# Autodesk Inventor assembly: Ensemble1
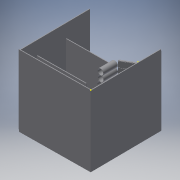
[picture p0: Inventor's stored thumbnail of the model, 180x180]
Saved by Autodesk Inventor 2019 (Build 230136000, 136)
## iProperties
Created: 2018-11-20
Part Number: Ensemble1
Material: Générique
Document SubType Name: Assembly
Designer: pouey
Author: pouey
## Documents named in this file (6)
- C:\Users\pouey\Desktop\PROJET ARDUINO\Ensemble1.iam
- C:\Users\pouey\Desktop\PROJET ARDUINO\boite.ipt
- C:\Users\pouey\Desktop\PROJET ARDUINO\V1.0_11-18.ipt
- C:\Users\pouey\Desktop\PROJET ARDUINO\planche.ipt
- C:\Users\pouey\Desktop\PROJET ARDUINO\toboggan.ipt
- C:\Users\pouey\Desktop\PROJET ARDUINO\tube.ipt
## Components (11 placed, 5 different names)
1. boite:1 — Placage:2, Placage:3, Placage:6, Placage:9, Placage:10, Placage:12, Placage:13, Placage:15, Placage:16, Placage:18, Angle:1
2. V1.0_11-18:1 — Placage:15, Placage:16
3. planche:1 — Placage:2, Placage:3, Placage:10, Placage:11
4. planche:2 — Placage:6, Placage:9, Placage:11, Placage:14
5. planche:3 — Placage:12, Placage:13, Placage:14
6. toboggan:1 — Placage:18, Angle:1, Placage:19, Placage:20, Placage:21, Placage:22, Placage:23
7. tube:1 — Placage:19
8. tube:2 — Placage:20
9. tube:3 — Placage:21
10. tube:4 — Placage:22
11. tube:5 — Placage:23
## Relationships (18: Mate 17, Angle 1)
- Placage:2 [Mate]: boite:1 ↔ planche:1
- Placage:3 [Mate] (120 mm): boite:1 ↔ planche:1
- Placage:6 [Mate]: boite:1 ↔ planche:2
- Placage:9 [Mate]: boite:1 ↔ planche:2
- Placage:10 [Mate]: boite:1 ↔ planche:1
- Placage:11 [Mate] (200 mm): planche:1 ↔ planche:2
- Placage:12 [Mate]: boite:1 ↔ planche:3
- Placage:13 [Mate]: boite:1 ↔ planche:3
- Placage:14 [Mate]: planche:2 ↔ planche:3
- Placage:15 [Mate]: boite:1 ↔ V1.0_11-18:1
- Placage:16 [Mate] (280 mm): boite:1 ↔ V1.0_11-18:1
- Placage:18 [Mate] (280 mm): boite:1 ↔ toboggan:1
- Angle:1 (120 deg): boite:1 ↔ toboggan:1
- Placage:19 [Mate] (17 mm): toboggan:1 ↔ tube:1
- Placage:20 [Mate] (18 mm): toboggan:1 ↔ tube:2
- Placage:21 [Mate] (17 mm): toboggan:1 ↔ tube:3
- Placage:22 [Mate] (17 mm): toboggan:1 ↔ tube:4
- Placage:23 [Mate] (17 mm): toboggan:1 ↔ tube:5
